# Autodesk Inventor assembly: Self Balancing Robot
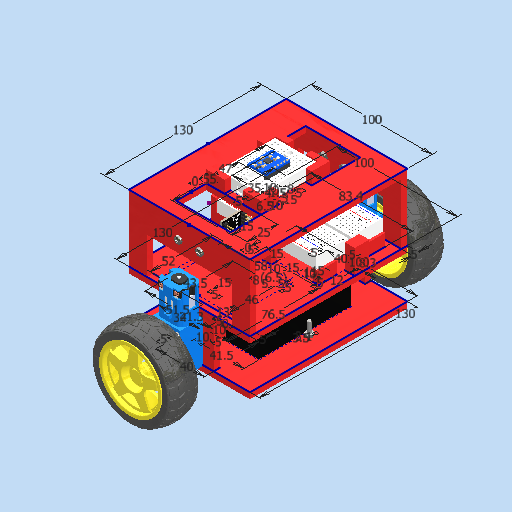
[picture p0: Inventor's stored thumbnail of the model, 512x512]
Saved by Autodesk Inventor 2026.2 (Build 302298010, 298A)
## iProperties
Created: 2025-12-05
Part Number: Self Balancing Robot
Document SubType Name: Assembly
Designer: maxim
Author: maxim
## Documents named in this file (16)
- C:\Users\maxim\OneDrive\Escritorio\Projects\Self Balancing Robot Project\Self Balancing Robot.iam
- C:\Users\maxim\Downloads\MPU6050 Module\MPU6050 Module\MPU6050 Module.ipt
- C:\Users\maxim\Downloads\ESP32Wroom32s\ESP32Wroom32s\ESP32Wroom32s.ipt
- C:\Users\maxim\Downloads\HalfBreadboard\HalfBreadboard\HalfBreadboard.ipt
- C:\Users\maxim\OneDrive\Escritorio\Projects\Self Balancing Robot Project\Baterías.ipt
- C:\Users\maxim\Downloads\Wheel D65x25 (1)\Wheel D65x25 (1)\Wheel D65x25 (1).ipt
- C:\Users\maxim\OneDrive\Escritorio\Projects\Self Balancing Robot Project\Chasis 1.ipt
- C:\Users\maxim\OneDrive\Escritorio\Projects\Self Balancing Robot Project\Chasis 2.ipt
- C:\Users\maxim\OneDrive\Escritorio\Projects\Self Balancing Robot Project\Chasis 3.ipt
- C:\Users\maxim\OneDrive\Documentos\Inventor\Content Center Files\R2025\en-US\AS 1427(05)\AS 1427 - M3 x 16(5) II.ipt
- C:\Users\maxim\OneDrive\Documentos\Inventor\Content Center Files\R2025\en-US\AS 1112 (2)\AS 1112 - M3  Type 5.ipt
- C:\Users\maxim\OneDrive\Documentos\Inventor\Content Center Files\R2025\en-US\AS 1427(05)\AS 1427 - M3 x 35(5) II.ipt
- C:\Users\maxim\Downloads\HW-411\HW-411\HW-411.ipt
- C:\Users\maxim\Downloads\Mini-White\Mini-White\Mini-White.ipt
- C:\Users\maxim\Downloads\tt-gearmotor-dc-3-6v-motorreductor-tt-high-precision-1.snapshot.1\MirlonJara_TT_Gearmotor_Metal_Blue_1Shaft_v1\01_Native_Files\TT_Gearmotor_Metal_Blue_2023\TT_Gearmotor_Metal_Blue_2023.ipt
- C:\Users\maxim\OneDrive\Escritorio\Projects\Self Balancing Robot Project\drv8833-doble-puente-h-dual-h-bridge-motor-driver-1.snapshot.3\Modulo DRV8833\Modulo_DRV8833_A\Modulo_DRV8833_A\Modulo_DRV8833_A.ipt
## Components (32 placed, 15 different names)
1. MPU6050 Module:1 — Mate:64
2. ESP32Wroom32s:1 — Mate:101, Mate:102
3. Wheel D65x25 (1):1 — Rotation:1, Mate:129, Mate:135
4. Wheel D65x25 (1):3 — Rotation:1, Mate:136, Mate:137, Mate:138
5. Chasis 1:1 — Mate:5, Mate:6, Mate:7, Mate:108, Mate:113, Mate:114, Mate:115, Mate:116, Mate:117, Mate:118, Mate:119, Mate:120, Mate:121, Mate:123, Mate:125
6. Chasis 2:1 — Mate:5, Mate:6, Mate:7, Mate:27, Mate:28, Mate:29, Mate:34, Mate:35, Mate:36, Mate:37, Mate:38, Mate:39, Mate:40, Mate:41, Mate:65, Mate:68, Mate:69, Mate:71, Mate:72, Mate:75, Mate:76, Mate:77, Mate:98, Mate:99, Mate:100, Mate:130
7. Chasis 3:1 — Mate:27, Mate:28, Mate:29, Mate:47, Mate:48, Mate:51, Mate:52, Mate:61, Mate:62, Mate:63
8. HalfBreadboard:2 — Mate:98, Mate:99, Mate:100, Mate:101, Mate:102
9. Mini-White:1 — Mate:61, Mate:62, Mate:63, Mate:64
10. AS 1427 H - Metric M3 x 16:1 — Mate:34, Mate:35, Mate:46
11. AS 1427 H - Metric M3 x 16:2 — Mate:36, Mate:37, Mate:49
12. AS 1427 H - Metric M3 x 16:3 — Mate:38, Mate:41, Mate:50
13. AS 1427 H - Metric M3 x 16:4 — Mate:39, Mate:40, Mate:53
14. AS 1427 H - Metric M3 x 35:1 — Mate:67, Mate:128, Mate:130, Mate:133
15. AS 1427 H - Metric M3 x 35:2 — Mate:65, Mate:70, Mate:124, Mate:134
16. AS 1427 H - Metric M3 x 35:3 — Mate:71, Mate:79, Mate:126, Mate:132
17. AS 1427 H - Metric M3 x 35:4 — Mate:72, Mate:78, Mate:127, Mate:131
18. AS 1112 (2) - Metric M3  Type 5:1 — Mate:46, Mate:47
19. AS 1112 (2) - Metric M3  Type 5:2 — Mate:48, Mate:49
20. AS 1112 (2) - Metric M3  Type 5:3 — Mate:50, Mate:51
21. AS 1112 (2) - Metric M3  Type 5:4 — Mate:52, Mate:53
22. AS 1112 (2) - Metric M3  Type 5:5 — Mate:67, Mate:68
23. AS 1112 (2) - Metric M3  Type 5:6 — Mate:69, Mate:70
24. AS 1112 (2) - Metric M3  Type 5:7 — Mate:75, Mate:77, Mate:78
25. AS 1112 (2) - Metric M3  Type 5:9 — Mate:76, Mate:79
26. AS 1112 (2) - Metric M3  Type 5:10 — Mate:108, Mate:121, Mate:122
27. AS 1427 H - Metric M3 x 16:5 — Mate:113, Mate:114, Mate:122
28. Baterías:1 — Mate:115, Mate:116, Mate:117
29. HW-411:1 — Mate:118, Mate:119, Mate:120
30. TT_Gearmotor_Metal_Blue_2023:1 — Mate:123, Mate:124, Mate:128, Mate:129, Mate:133, Mate:134, Mate:135
31. TT_Gearmotor_Metal_Blue_2023:2 — Mate:125, Mate:126, Mate:127, Mate:131, Mate:132, Mate:136, Mate:137, Mate:138
32. Modulo_DRV8833_A:1
## Relationships (71: Mate 70, RelateRotation 1)
- Mate:5: Chasis 1:1 ↔ Chasis 2:1
- Mate:6: Chasis 1:1 ↔ Chasis 2:1
- Mate:7: Chasis 1:1 ↔ Chasis 2:1
- Rotation:1 [RelateRotation] (1 ul): Wheel D65x25 (1):1 ↔ Wheel D65x25 (1):3
- Mate:27: Chasis 2:1 ↔ Chasis 3:1
- Mate:28: Chasis 2:1 ↔ Chasis 3:1
- Mate:29: Chasis 2:1 ↔ Chasis 3:1
- Mate:34: Chasis 2:1 ↔ AS 1427 H - Metric M3 x 16:1
- Mate:35: Chasis 2:1 ↔ AS 1427 H - Metric M3 x 16:1
- Mate:36: Chasis 2:1 ↔ AS 1427 H - Metric M3 x 16:2
- Mate:37: Chasis 2:1 ↔ AS 1427 H - Metric M3 x 16:2
- Mate:38: Chasis 2:1 ↔ AS 1427 H - Metric M3 x 16:3
- Mate:39: Chasis 2:1 ↔ AS 1427 H - Metric M3 x 16:4
- Mate:40: Chasis 2:1 ↔ AS 1427 H - Metric M3 x 16:4
- Mate:41: Chasis 2:1 ↔ AS 1427 H - Metric M3 x 16:3
- Mate:46: AS 1427 H - Metric M3 x 16:1 ↔ AS 1112 (2) - Metric M3  Type 5:1
- Mate:47: Chasis 3:1 ↔ AS 1112 (2) - Metric M3  Type 5:1
- Mate:48: Chasis 3:1 ↔ AS 1112 (2) - Metric M3  Type 5:2
- Mate:49: AS 1427 H - Metric M3 x 16:2 ↔ AS 1112 (2) - Metric M3  Type 5:2
- Mate:50: AS 1427 H - Metric M3 x 16:3 ↔ AS 1112 (2) - Metric M3  Type 5:3
- Mate:51: Chasis 3:1 ↔ AS 1112 (2) - Metric M3  Type 5:3
- Mate:52: Chasis 3:1 ↔ AS 1112 (2) - Metric M3  Type 5:4
- Mate:53: AS 1427 H - Metric M3 x 16:4 ↔ AS 1112 (2) - Metric M3  Type 5:4
- Mate:61: Chasis 3:1 ↔ Mini-White:1
- Mate:62: Chasis 3:1 ↔ Mini-White:1
- Mate:63: Chasis 3:1 ↔ Mini-White:1
- Mate:64: MPU6050 Module:1 ↔ Mini-White:1
- Mate:65: Chasis 2:1 ↔ AS 1427 H - Metric M3 x 35:2
- Mate:67: AS 1427 H - Metric M3 x 35:1 ↔ AS 1112 (2) - Metric M3  Type 5:5
- Mate:68: Chasis 2:1 ↔ AS 1112 (2) - Metric M3  Type 5:5
- Mate:69: Chasis 2:1 ↔ AS 1112 (2) - Metric M3  Type 5:6
- Mate:70: AS 1427 H - Metric M3 x 35:2 ↔ AS 1112 (2) - Metric M3  Type 5:6
- Mate:71: Chasis 2:1 ↔ AS 1427 H - Metric M3 x 35:3
- Mate:72: Chasis 2:1 ↔ AS 1427 H - Metric M3 x 35:4
- Mate:75: Chasis 2:1 ↔ AS 1112 (2) - Metric M3  Type 5:7
- Mate:76: Chasis 2:1 ↔ AS 1112 (2) - Metric M3  Type 5:9
- Mate:77: Chasis 2:1 ↔ AS 1112 (2) - Metric M3  Type 5:7
- Mate:78: AS 1427 H - Metric M3 x 35:4 ↔ AS 1112 (2) - Metric M3  Type 5:7
- Mate:79: AS 1427 H - Metric M3 x 35:3 ↔ AS 1112 (2) - Metric M3  Type 5:9
- Mate:98: Chasis 2:1 ↔ HalfBreadboard:2
- Mate:99: Chasis 2:1 ↔ HalfBreadboard:2
- Mate:100: Chasis 2:1 ↔ HalfBreadboard:2
- Mate:101: ESP32Wroom32s:1 ↔ HalfBreadboard:2
- Mate:102: ESP32Wroom32s:1 ↔ HalfBreadboard:2
- Mate:108: Chasis 1:1 ↔ AS 1112 (2) - Metric M3  Type 5:10
- Mate:113: Chasis 1:1 ↔ AS 1427 H - Metric M3 x 16:5
- Mate:114: Chasis 1:1 ↔ AS 1427 H - Metric M3 x 16:5
- Mate:115: Chasis 1:1 ↔ Baterías:1
- Mate:116: Chasis 1:1 ↔ Baterías:1
- Mate:117: Chasis 1:1 ↔ Baterías:1
- Mate:118: Chasis 1:1 ↔ HW-411:1
- Mate:119: Chasis 1:1 ↔ HW-411:1
- Mate:120: Chasis 1:1 ↔ HW-411:1
- Mate:121: Chasis 1:1 ↔ AS 1112 (2) - Metric M3  Type 5:10
- Mate:122: AS 1112 (2) - Metric M3  Type 5:10 ↔ AS 1427 H - Metric M3 x 16:5
- Mate:123: Chasis 1:1 ↔ TT_Gearmotor_Metal_Blue_2023:1
- Mate:124: AS 1427 H - Metric M3 x 35:2 ↔ TT_Gearmotor_Metal_Blue_2023:1
- Mate:125: Chasis 1:1 ↔ TT_Gearmotor_Metal_Blue_2023:2
- Mate:126: AS 1427 H - Metric M3 x 35:3 ↔ TT_Gearmotor_Metal_Blue_2023:2
- Mate:127: AS 1427 H - Metric M3 x 35:4 ↔ TT_Gearmotor_Metal_Blue_2023:2
- Mate:128: AS 1427 H - Metric M3 x 35:1 ↔ TT_Gearmotor_Metal_Blue_2023:1
- Mate:129: Wheel D65x25 (1):1 ↔ TT_Gearmotor_Metal_Blue_2023:1
- Mate:130: Chasis 2:1 ↔ AS 1427 H - Metric M3 x 35:1
- Mate:131: AS 1427 H - Metric M3 x 35:4 ↔ TT_Gearmotor_Metal_Blue_2023:2
- Mate:132: AS 1427 H - Metric M3 x 35:3 ↔ TT_Gearmotor_Metal_Blue_2023:2
- Mate:133: AS 1427 H - Metric M3 x 35:1 ↔ TT_Gearmotor_Metal_Blue_2023:1
- Mate:134: AS 1427 H - Metric M3 x 35:2 ↔ TT_Gearmotor_Metal_Blue_2023:1
- Mate:135: Wheel D65x25 (1):1 ↔ TT_Gearmotor_Metal_Blue_2023:1
- Mate:136: Wheel D65x25 (1):3 ↔ TT_Gearmotor_Metal_Blue_2023:2
- Mate:137: Wheel D65x25 (1):3 ↔ TT_Gearmotor_Metal_Blue_2023:2
- Mate:138: Wheel D65x25 (1):3 ↔ TT_Gearmotor_Metal_Blue_2023:2
